# Autodesk Inventor assembly: servocheck
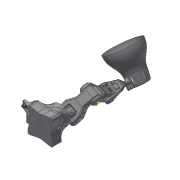
[picture p0: Inventor's stored thumbnail of the model, 180x180]
Saved by Autodesk Inventor 2018 (Build 220112000, 112)
## iProperties
Created: 2018-02-01
Part Number: servocheck
Document SubType Name: Assembly
Designer: Clevo
Author: Clevo
## Documents named in this file (29)
- E:\RobotArm\MCAD\servocheck.iam
- E:\RobotArm\MCAD\LX-16A.iam
- E:\RobotArm\MCAD\base.ipt
- E:\RobotArm\MCAD\52407bearing.ipt
- E:\RobotArm\MCAD\table.ipt
- E:\RobotArm\MCAD\arm2.ipt
- E:\RobotArm\MCAD\arm2bearing_carrier.ipt
- E:\RobotArm\MCAD\armbearing1.ipt
- E:\RobotArm\MCAD\arm3.ipt
- E:\RobotArm\MCAD\arm4.ipt
- E:\RobotArm\MCAD\c_axisrot.ipt
- E:\RobotArm\MCAD\bottomarm.iam
- E:\RobotArm\MCAD\basebtm.ipt
- E:\RobotArm\MCAD\arm6vers2.ipt
- E:\RobotArm\MCAD\MG90servo_assembly.iam
- E:\RobotArm\MCAD\91274A141_COATED ALLOY STEEL SOCKET HEAD CAP SCREW.ipt
- E:\RobotArm\MCAD\91292A027_TYPE 18-8 SS SOCKET HEAD CAP SCREW.ipt
- E:\RobotArm\MCAD\91292A123_TYPE 18-8 SS SOCKET HEAD CAP SCREW.ipt
- E:\RobotArm\MCAD\91292A831_TYPE 18-8 SS SOCKET HEAD CAP SCREW.ipt
- E:\RobotArm\MCAD\base_filler.ipt
- E:\RobotArm\MCAD\test_tip.ipt
- E:\RobotArm\MCAD\filesforprint\FakeGripper.ipt
- E:\RobotArm\MCAD\baseclamp.ipt
- E:\RobotArm\MCAD\Lamp_Shade.ipt
- E:\RobotArm\MCAD\Light_Base.ipt
- E:\RobotArm\MCAD\Camera_Assem.iam
- E:\RobotArm\MCAD\Switch_Panel.ipt
- E:\RobotArm\MCAD\miniature-toggle-switch-1.snapshot.1\Eledis 1A11-NF1STSE SPDT Toggle Switch.ipt
- E:\RobotArm\MCAD\Switch_Extend.ipt
## Components (51 placed, 28 different names)
1. LX-16A:1 [sub-assembly] — Mate:3, Mate:4, Angle:1, Mate:8
2. base:1 — Mate:3, Mate:4, Angle:1, Mate:5, Mate:6, Mate:52, Mate:53, Mate:54, Mate:82, Mate:83, Mate:84, Mate:85, Mate:86, Mate:87, Mate:88, Mate:89, Flush:5, Mate:107, Mate:114, Angle:14
3. 52407bearing:1 — Mate:5, Mate:6, Mate:7, Mate:106
4. table:1 — Mate:7, Mate:8, Mate:46, Mate:47, Mate:48
5. LX-16A:3 [sub-assembly] — Mate:18, Mate:19, Mate:41, Angle:11, Mate:51
6. arm2:1 — Mate:18, Mate:19, Mate:20, Mate:21, Mate:22, Mate:31, Mate:32, Angle:11, Mate:51
7. arm2bearing_carrier:1 — Mate:20, Mate:21, Mate:22, Mate:23, Mate:24, Angle:12
8. armbearing1:1 — Mate:23, Mate:24, Mate:38
9. LX-16A:4 [sub-assembly] — Mate:35, Mate:36, Angle:8
10. arm4:1 — Mate:28, Mate:29, Angle:6, Mate:31, Mate:32, Mate:49, Mate:50, Mate:98, Mate:99, Mate:100, Mate:101, Mate:102, Mate:103, Mate:104, Mate:105
11. LX-16A:5 [sub-assembly] — Mate:28, Mate:29, Angle:6
12. LX-16A:6 [sub-assembly] — Mate:55, Mate:56, Angle:13, Mate:109, Mate:110
13. arm3:1 — Mate:35, Mate:36, Angle:8, Mate:44, Mate:45, Flush:4, Angle:12, Mate:57, Mate:58
14. c_axisrot:1 — Mate:38, Mate:41, Mate:44, Mate:45, Flush:4
15. bottomarm:1 [sub-assembly] — Mate:46, Mate:47, Mate:48, Mate:49, Mate:50, Angle:10, Mate:59, Mate:60, Mate:61, Mate:62, Mate:64, Mate:67, Mate:68, Mate:69, Mate:70, Mate:71, Mate:72, Mate:73, Mate:74, Mate:75, Mate:76, Mate:77, Mate:78, Mate:79, Mate:80, Mate:81, Mate:90, Mate:91, Mate:92, Mate:93, Mate:94, Mate:95, Mate:96, Mate:97
16. basebtm:1 — Mate:52, Mate:53, Mate:54
17. arm6vers2:1 — Mate:55, Mate:56, Angle:13, Mate:57, Mate:58, Mate:108
18. MG90servo_assembly:1 [sub-assembly]
19. MG90servo_assembly:2 [sub-assembly]
20. 91274A141_COATED ALLOY STEEL SOCKET HEAD CAP SCREW:1 — Mate:82, Mate:88
21. 91292A831_TYPE 18-8 SS SOCKET HEAD CAP SCREW:2 — Mate:59, Mate:68
22. 91292A831_TYPE 18-8 SS SOCKET HEAD CAP SCREW:3 — Mate:62, Mate:70
23. 91292A831_TYPE 18-8 SS SOCKET HEAD CAP SCREW:4 — Mate:61, Mate:69
24. 91292A831_TYPE 18-8 SS SOCKET HEAD CAP SCREW:5 — Mate:60, Mate:67
25. 91292A831_TYPE 18-8 SS SOCKET HEAD CAP SCREW:9 — Mate:64, Mate:77
26. 91292A831_TYPE 18-8 SS SOCKET HEAD CAP SCREW:10 — Mate:71, Mate:76
27. 91292A831_TYPE 18-8 SS SOCKET HEAD CAP SCREW:11 — Mate:72, Mate:75
28. 91292A831_TYPE 18-8 SS SOCKET HEAD CAP SCREW:12 — Mate:73, Mate:74
29. 91292A123_TYPE 18-8 SS SOCKET HEAD CAP SCREW:2 — Mate:78, Mate:79
30. 91292A123_TYPE 18-8 SS SOCKET HEAD CAP SCREW:3 — Mate:80, Mate:81
31. 91274A141_COATED ALLOY STEEL SOCKET HEAD CAP SCREW:2 — Mate:83, Mate:89
32. 91274A141_COATED ALLOY STEEL SOCKET HEAD CAP SCREW:3 — Mate:85, Mate:86, Mate:115
33. 91274A141_COATED ALLOY STEEL SOCKET HEAD CAP SCREW:4 — Mate:84, Mate:87, Mate:116
34. 91292A027_TYPE 18-8 SS SOCKET HEAD CAP SCREW:2 — Mate:90, Mate:94
35. 91292A027_TYPE 18-8 SS SOCKET HEAD CAP SCREW:3 — Mate:91, Mate:96
36. 91292A027_TYPE 18-8 SS SOCKET HEAD CAP SCREW:4 — Mate:93, Mate:95
37. 91292A027_TYPE 18-8 SS SOCKET HEAD CAP SCREW:5 — Mate:92, Mate:97
38. 91292A027_TYPE 18-8 SS SOCKET HEAD CAP SCREW:6 — Mate:98, Mate:102
39. 91292A027_TYPE 18-8 SS SOCKET HEAD CAP SCREW:7 — Mate:101, Mate:103
40. 91292A027_TYPE 18-8 SS SOCKET HEAD CAP SCREW:8 — Mate:99, Mate:105
41. 91292A027_TYPE 18-8 SS SOCKET HEAD CAP SCREW:9 — Mate:100, Mate:104
42. base_filler:1 — Flush:5, Mate:106, Mate:107
43. test_tip:1 — Mate:108, Mate:109, Mate:110, Mate:111, Mate:112, Mate:113, Mate:117, Mate:118
44. FakeGripper:1 — Mate:111, Mate:112, Mate:113
45. baseclamp:1 — Mate:114, Mate:115, Mate:116, Mate:123, Flush:6
46. Lamp_Shade:1 — Mate:117, Mate:118, Mate:119, Tangent:1, Angle:16
47. Light_Base:1 — Mate:119, Tangent:1, Mate:120, Mate:121, Mate:122, Angle:16
48. Camera_Assem:1 [sub-assembly] — Mate:120, Mate:121, Mate:122
49. Switch_Panel:1 — Mate:123, Flush:6, Angle:14, Mate:124, Mate:125, Angle:15, Mate:127
50. Eledis 1A11-NF1STSE SPDT Toggle Switch:1 — Mate:124, Mate:125, Angle:15, Mate:126
51. Switch_Extend:1 — Mate:126, Mate:127
## Relationships (116: Mate 102, Angle 10, Flush 3, Tangent 1)
- Mate:3: LX-16A:1 ↔ base:1
- Mate:4: LX-16A:1 ↔ base:1
- Angle:1 (270 deg): LX-16A:1 ↔ base:1
- Mate:5: base:1 ↔ 52407bearing:1
- Mate:6: base:1 ↔ 52407bearing:1
- Mate:7: 52407bearing:1 ↔ table:1
- Mate:8: LX-16A:1 ↔ table:1
- Mate:18: LX-16A:3 ↔ arm2:1
- Mate:19: LX-16A:3 ↔ arm2:1
- Mate:20: arm2:1 ↔ arm2bearing_carrier:1
- Mate:21: arm2:1 ↔ arm2bearing_carrier:1
- Mate:22: arm2:1 ↔ arm2bearing_carrier:1
- Mate:23: arm2bearing_carrier:1 ↔ armbearing1:1
- Mate:24: arm2bearing_carrier:1 ↔ armbearing1:1
- Mate:28: arm4:1 ↔ LX-16A:5
- Mate:29: arm4:1 ↔ LX-16A:5
- Angle:6 (90 deg): arm4:1 ↔ LX-16A:5
- Mate:31: arm2:1 ↔ arm4:1
- Mate:32 (0.25 mm): arm2:1 ↔ arm4:1
- Mate:35: LX-16A:4 ↔ arm3:1
- Mate:36: LX-16A:4 ↔ arm3:1
- Angle:8 (0 deg): LX-16A:4 ↔ arm3:1
- Mate:38: armbearing1:1 ↔ c_axisrot:1
- Mate:41: LX-16A:3 ↔ c_axisrot:1
- Mate:44 (0.05 mm): arm3:1 ↔ c_axisrot:1
- Mate:45 (0.05 mm): arm3:1 ↔ c_axisrot:1
- Flush:4: arm3:1 ↔ c_axisrot:1
- Mate:46: table:1 ↔ bottomarm:1
- Mate:47: table:1 ↔ bottomarm:1
- Mate:48: table:1 ↔ bottomarm:1
- Mate:49: arm4:1 ↔ bottomarm:1
- Mate:50: arm4:1 ↔ bottomarm:1
- Angle:10 (0 deg): bottomarm:1
- Angle:11 (270 deg): LX-16A:3 ↔ arm2:1
- Mate:51 (0.0883 mm): LX-16A:3 ↔ arm2:1
- Mate:52: base:1 ↔ basebtm:1
- Mate:53: base:1 ↔ basebtm:1
- Mate:54: base:1 ↔ basebtm:1
- Angle:12 (0 deg): arm2bearing_carrier:1 ↔ arm3:1
- Mate:55: LX-16A:6 ↔ arm6vers2:1
- Mate:56: LX-16A:6 ↔ arm6vers2:1
- Angle:13 (-90 deg): LX-16A:6 ↔ arm6vers2:1
- Mate:57: arm3:1 ↔ arm6vers2:1
- Mate:58 (0.25 mm): arm3:1 ↔ arm6vers2:1
- Mate:59: bottomarm:1 ↔ 91292A831_TYPE 18-8 SS SOCKET HEAD CAP SCREW:2
- Mate:60: bottomarm:1 ↔ 91292A831_TYPE 18-8 SS SOCKET HEAD CAP SCREW:5
- Mate:61: bottomarm:1 ↔ 91292A831_TYPE 18-8 SS SOCKET HEAD CAP SCREW:4
- Mate:62: bottomarm:1 ↔ 91292A831_TYPE 18-8 SS SOCKET HEAD CAP SCREW:3
- Mate:64: bottomarm:1 ↔ 91292A831_TYPE 18-8 SS SOCKET HEAD CAP SCREW:9
- Mate:67: bottomarm:1 ↔ 91292A831_TYPE 18-8 SS SOCKET HEAD CAP SCREW:5
- Mate:68: bottomarm:1 ↔ 91292A831_TYPE 18-8 SS SOCKET HEAD CAP SCREW:2
- Mate:69: bottomarm:1 ↔ 91292A831_TYPE 18-8 SS SOCKET HEAD CAP SCREW:4
- Mate:70: bottomarm:1 ↔ 91292A831_TYPE 18-8 SS SOCKET HEAD CAP SCREW:3
- Mate:71: bottomarm:1 ↔ 91292A831_TYPE 18-8 SS SOCKET HEAD CAP SCREW:10
- Mate:72: bottomarm:1 ↔ 91292A831_TYPE 18-8 SS SOCKET HEAD CAP SCREW:11
- Mate:73: bottomarm:1 ↔ 91292A831_TYPE 18-8 SS SOCKET HEAD CAP SCREW:12
- Mate:74: bottomarm:1 ↔ 91292A831_TYPE 18-8 SS SOCKET HEAD CAP SCREW:12
- Mate:75: bottomarm:1 ↔ 91292A831_TYPE 18-8 SS SOCKET HEAD CAP SCREW:11
- Mate:76: bottomarm:1 ↔ 91292A831_TYPE 18-8 SS SOCKET HEAD CAP SCREW:10
- Mate:77: bottomarm:1 ↔ 91292A831_TYPE 18-8 SS SOCKET HEAD CAP SCREW:9
- Mate:78: bottomarm:1 ↔ 91292A123_TYPE 18-8 SS SOCKET HEAD CAP SCREW:2
- Mate:79: bottomarm:1 ↔ 91292A123_TYPE 18-8 SS SOCKET HEAD CAP SCREW:2
- Mate:80: bottomarm:1 ↔ 91292A123_TYPE 18-8 SS SOCKET HEAD CAP SCREW:3
- Mate:81: bottomarm:1 ↔ 91292A123_TYPE 18-8 SS SOCKET HEAD CAP SCREW:3
- Mate:82: base:1 ↔ 91274A141_COATED ALLOY STEEL SOCKET HEAD CAP SCREW:1
- Mate:83: base:1 ↔ 91274A141_COATED ALLOY STEEL SOCKET HEAD CAP SCREW:2
- Mate:84: base:1 ↔ 91274A141_COATED ALLOY STEEL SOCKET HEAD CAP SCREW:4
- Mate:85: base:1 ↔ 91274A141_COATED ALLOY STEEL SOCKET HEAD CAP SCREW:3
- Mate:86: base:1 ↔ 91274A141_COATED ALLOY STEEL SOCKET HEAD CAP SCREW:3
- Mate:87: base:1 ↔ 91274A141_COATED ALLOY STEEL SOCKET HEAD CAP SCREW:4
- Mate:88: base:1 ↔ 91274A141_COATED ALLOY STEEL SOCKET HEAD CAP SCREW:1
- Mate:89: base:1 ↔ 91274A141_COATED ALLOY STEEL SOCKET HEAD CAP SCREW:2
- Mate:90: bottomarm:1 ↔ 91292A027_TYPE 18-8 SS SOCKET HEAD CAP SCREW:2
- Mate:91: bottomarm:1 ↔ 91292A027_TYPE 18-8 SS SOCKET HEAD CAP SCREW:3
- Mate:92: bottomarm:1 ↔ 91292A027_TYPE 18-8 SS SOCKET HEAD CAP SCREW:5
- Mate:93: bottomarm:1 ↔ 91292A027_TYPE 18-8 SS SOCKET HEAD CAP SCREW:4
- Mate:94: bottomarm:1 ↔ 91292A027_TYPE 18-8 SS SOCKET HEAD CAP SCREW:2
- Mate:95: bottomarm:1 ↔ 91292A027_TYPE 18-8 SS SOCKET HEAD CAP SCREW:4
- Mate:96: bottomarm:1 ↔ 91292A027_TYPE 18-8 SS SOCKET HEAD CAP SCREW:3
- Mate:97: bottomarm:1 ↔ 91292A027_TYPE 18-8 SS SOCKET HEAD CAP SCREW:5
- Mate:98: arm4:1 ↔ 91292A027_TYPE 18-8 SS SOCKET HEAD CAP SCREW:6
- Mate:99: arm4:1 ↔ 91292A027_TYPE 18-8 SS SOCKET HEAD CAP SCREW:8
- Mate:100: arm4:1 ↔ 91292A027_TYPE 18-8 SS SOCKET HEAD CAP SCREW:9
- Mate:101: arm4:1 ↔ 91292A027_TYPE 18-8 SS SOCKET HEAD CAP SCREW:7
- Mate:102: arm4:1 ↔ 91292A027_TYPE 18-8 SS SOCKET HEAD CAP SCREW:6
- Mate:103: arm4:1 ↔ 91292A027_TYPE 18-8 SS SOCKET HEAD CAP SCREW:7
- Mate:104: arm4:1 ↔ 91292A027_TYPE 18-8 SS SOCKET HEAD CAP SCREW:9
- Mate:105: arm4:1 ↔ 91292A027_TYPE 18-8 SS SOCKET HEAD CAP SCREW:8
- Flush:5: base:1 ↔ base_filler:1
- Mate:106: 52407bearing:1 ↔ base_filler:1
- Mate:107: base:1 ↔ base_filler:1
- Mate:108: arm6vers2:1 ↔ test_tip:1
- Mate:109: LX-16A:6 ↔ test_tip:1
- Mate:110: LX-16A:6 ↔ test_tip:1
- Mate:111: test_tip:1 ↔ FakeGripper:1
- Mate:112: test_tip:1 ↔ FakeGripper:1
- Mate:113: test_tip:1 ↔ FakeGripper:1
- Mate:114: base:1 ↔ baseclamp:1
- Mate:115: 91274A141_COATED ALLOY STEEL SOCKET HEAD CAP SCREW:3 ↔ baseclamp:1
- Mate:116: 91274A141_COATED ALLOY STEEL SOCKET HEAD CAP SCREW:4 ↔ baseclamp:1
- Mate:117: test_tip:1 ↔ Lamp_Shade:1
- Mate:118: test_tip:1 ↔ Lamp_Shade:1
- Mate:119: Lamp_Shade:1 ↔ Light_Base:1
- Tangent:1: Lamp_Shade:1 ↔ Light_Base:1
- Mate:120: Light_Base:1 ↔ Camera_Assem:1
- Mate:121: Light_Base:1 ↔ Camera_Assem:1
- Mate:122: Light_Base:1 ↔ Camera_Assem:1
- Mate:123: baseclamp:1 ↔ Switch_Panel:1
- Flush:6: baseclamp:1 ↔ Switch_Panel:1
- Angle:14 (180 deg): base:1 ↔ Switch_Panel:1
- Mate:124: Switch_Panel:1 ↔ Eledis 1A11-NF1STSE SPDT Toggle Switch:1
- Mate:125: Switch_Panel:1 ↔ Eledis 1A11-NF1STSE SPDT Toggle Switch:1
- Angle:15 (0 deg): Switch_Panel:1 ↔ Eledis 1A11-NF1STSE SPDT Toggle Switch:1
- Mate:126: Eledis 1A11-NF1STSE SPDT Toggle Switch:1 ↔ Switch_Extend:1
- Mate:127 (-11 mm): Switch_Panel:1 ↔ Switch_Extend:1
- Angle:16 (0 deg): Lamp_Shade:1 ↔ Light_Base:1
